# Autodesk Inventor assembly: Assembly1
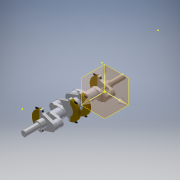
[picture p0: Inventor's stored thumbnail of the model, 180x180]
Saved by Autodesk Inventor 2019 (Build 230136000, 136)
## iProperties
Created: 2019-06-29
Part Number: Assembly1
Document SubType Name: Assembly
Designer: usuario
Mass: 181.192 g
Surface Area: 482.745 cm^2
Volume: 172.255 cm^3
Density: 1.05188 g/cm^3
Author: usuario
## Documents named in this file (7)
- E:\OSCAR\UNAL\6to SEMESTRE\Principios de dinámica\Proyectos\Proyecto 2\Mio\Sin_Vibraciones.iam
- E:\OSCAR\UNAL\6to SEMESTRE\Principios de dinámica\Proyectos\Proyecto 2\Mio\cigueñal.ipt
- E:\OSCAR\UNAL\6to SEMESTRE\Principios de dinámica\Proyectos\Proyecto 2\Mio\Contrapeso2.ipt
- E:\OSCAR\UNAL\6to SEMESTRE\Principios de dinámica\Proyectos\Proyecto 2\Mio\Contrapeso1.ipt
- E:\OSCAR\UNAL\6to SEMESTRE\Principios de dinámica\Proyectos\Proyecto 2\Mio\Contrapeso4.ipt
- E:\OSCAR\UNAL\6to SEMESTRE\Principios de dinámica\Proyectos\Proyecto 2\Mio\Contrapeso5.ipt
- E:\OSCAR\UNAL\6to SEMESTRE\Principios de dinámica\Proyectos\Proyecto 2\Mio\Pasador 2.ipt
## Components (13 placed, 6 different names)
1. cigueñal:1 — Rigid:2, Rotational:1, Rotational:2, Rotational:3, Insert:1, Insert:3, Insert:6, Insert:7, Insert:8, Rigid:3
2. Contrapeso2:1 — Rigid:2, Insert:4, Insert:5
3. Contrapeso1:1 — Rotational:1
4. Contrapeso4:1 — Rotational:2, Rigid:3
5. Contrapeso5:1 — Rotational:3, Insert:2
6. Pasador 2:1 — Insert:3
7. Pasador 2:2 — Insert:4
8. Pasador 2:3 — Insert:1
9. Pasador 2:4 — Insert:2
10. Pasador 2:5 — Insert:8
11. Pasador 2:6 — Insert:7
12. Pasador 2:7 — Insert:5
13. Pasador 2:8 — Insert:6
## Relationships (13: Insert 8, RevoluteJoint 3, WeldJoint 2)
- Rigid:2 [WeldJoint]: cigueñal:1 ↔ Contrapeso2:1
- Rotational:1 [RevoluteJoint]: cigueñal:1 ↔ Contrapeso1:1
- Rotational:2 [RevoluteJoint]: cigueñal:1 ↔ Contrapeso4:1
- Rotational:3 [RevoluteJoint]: cigueñal:1 ↔ Contrapeso5:1
- Insert:1 (-9 mm): cigueñal:1 ↔ Pasador 2:3
- Insert:2 (-7 mm): Contrapeso5:1 ↔ Pasador 2:4
- Insert:3 (-9 mm): cigueñal:1 ↔ Pasador 2:1
- Insert:4 (-7 mm): Contrapeso2:1 ↔ Pasador 2:2
- Insert:5 (-7 mm): Contrapeso2:1 ↔ Pasador 2:7
- Insert:6 (-9 mm): cigueñal:1 ↔ Pasador 2:8
- Insert:7 (-9 mm): cigueñal:1 ↔ Pasador 2:6
- Insert:8 (-9 mm): cigueñal:1 ↔ Pasador 2:5
- Rigid:3 [WeldJoint]: cigueñal:1 ↔ Contrapeso4:1
